# Autodesk Inventor assembly: 60T厚齿轮带铁芯
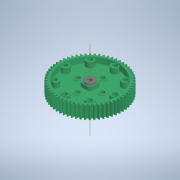
[picture p0: Inventor's stored thumbnail of the model, 180x180]
Saved by Autodesk Inventor 2020 (Build 240168000, 168)
## iProperties
Created: 2019-05-29
Part Number: 60T厚齿轮带铁芯
Document SubType Name: Assembly
Designer: aresp
Author: aresp
## Documents named in this file (3)
- D:\vault\ncrCadLib\齿轮\60T厚齿轮带铁芯.iam
- D:\vault\ncrCadLib\齿轮\Gear HS 60 tooth.ipt
- D:\vault\ncrCadLib\齿轮\Insert HS Metal.ipt
## Components (3 placed, 2 different names)
1. Gear HS 60 tooth:1 — 配合:1, 配合:2, 配合:3, 配合:4
2. Insert HS Metal:1 — 配合:1, 表面齐平:1, 配合:4
3. Insert HS Metal:2 — 配合:2, 配合:3, 表面齐平:1
## Relationships (5: Mate 4, Flush 1)
- 配合:1 [Mate]: Gear HS 60 tooth:1 ↔ Insert HS Metal:1
- 配合:2 [Mate]: Gear HS 60 tooth:1 ↔ Insert HS Metal:2
- 配合:3 [Mate]: Gear HS 60 tooth:1 ↔ Insert HS Metal:2
- 表面齐平:1 [Flush]: Insert HS Metal:1 ↔ Insert HS Metal:2
- 配合:4 [Mate]: Gear HS 60 tooth:1 ↔ Insert HS Metal:1
